# Autodesk Inventor assembly: PowerDistroAssembly_RevB
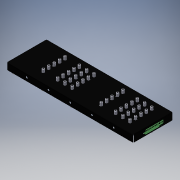
[picture p0: Inventor's stored thumbnail of the model, 180x180]
Saved by Autodesk Inventor 2018 (Build 220112000, 112)
## iProperties
Created: 2018-06-27
Part Number: PowerDistroAssembly_RevB
Document SubType Name: Assembly
Designer: Rich
Author: Rich
## Documents named in this file (8)
- C:\Users\Rich\development\UWaterloo\power-distro.git\SolidModels\PowerDistroAssembly_RevB.iam
- C:\Users\Rich\development\UWaterloo\power-distro.git\SolidModels\power_distro_pcb_RevB.ipt
- C:\Users\Rich\development\UWaterloo\power-distro.git\SolidModels\rcj-021.iam
- C:\Users\Rich\development\UWaterloo\power-distro.git\SolidModels\Enclosure2_RevB_Outer.ipt
- C:\Users\Rich\development\UWaterloo\power-distro.git\SolidModels\Enclosure2_RevB_Inner.ipt
- C:\Users\Rich\development\UWaterloo\power-distro.git\SolidModels\keystone-PN1608-2.ipt
- C:\Users\Rich\development\UWaterloo\power-distro.git\SolidModels\6-32x0.25 Slotted Flathead.ipt
- C:\Users\Rich\development\UWaterloo\power-distro.git\SolidModels\3_5mm_5_08mm_adapter_assembly.iam
## Components (77 placed, 7 different names)
1. power_distro_pcb_RevB:1 — Mate:1, Mate:2, Mate:3, Mate:4, Angle:6, Tangent:1, Mate:5, Angle:7, Mate:6, Mate:7, Mate:10, Mate:11, Mate:12, Mate:13, Mate:14, Mate:15, Mate:16, Mate:17, Mate:18, Mate:19, Mate:20, Mate:21, Mate:22, Mate:23, Mate:24, Mate:25, Mate:26, Mate:27, Insert:1, Insert:2, Insert:3, Insert:4, Insert:5, Insert:6, Insert:7, Insert:8, Insert:9, Mate:34, Mate:35, Mate:36, Mate:37, Mate:38, Mate:39
2. Enclosure2_RevB_Outer:1 — Mate:30, Mate:31, Mate:32
3. Enclosure2_RevB_Inner:2 — Mate:8, Mate:9, Mate:28, Mate:30, Insert:10, Mate:33
4. keystone-PN1608-2:1 — Mate:6, Mate:7, Mate:8, Mate:9
5. keystone-PN1608-2:2 — Mate:10, Mate:27
6. keystone-PN1608-2:3 — Mate:15, Mate:21, Mate:28, Mate:29
7. keystone-PN1608-2:4 — Mate:16, Mate:20
8. keystone-PN1608-2:5 — Mate:11, Mate:25
9. keystone-PN1608-2:6 — Mate:18, Mate:19
10. keystone-PN1608-2:7 — Mate:17, Mate:22
11. keystone-PN1608-2:8 — Mate:14, Mate:26
12. keystone-PN1608-2:9 — Mate:13, Mate:23
13. keystone-PN1608-2:10 — Mate:12, Mate:24
14. 6-32x0.25 Slotted Flathead:1 — Mate:29
15. 6-32x0.25 Slotted Flathead:2 — Insert:1
16. 6-32x0.25 Slotted Flathead:3 — Insert:6
17. 6-32x0.25 Slotted Flathead:4 — Insert:7
18. 6-32x0.25 Slotted Flathead:5 — Insert:8
19. 6-32x0.25 Slotted Flathead:6 — Insert:9
20. 6-32x0.25 Slotted Flathead:7 — Insert:5
21. 6-32x0.25 Slotted Flathead:8 — Insert:4
22. 6-32x0.25 Slotted Flathead:9 — Insert:3
23. 6-32x0.25 Slotted Flathead:10 — Insert:2
24. 6-32x0.25 Slotted Flathead:11
25. 6-32x0.25 Slotted Flathead:12
26. 6-32x0.25 Slotted Flathead:13
27. 6-32x0.25 Slotted Flathead:14
28. 6-32x0.25 Slotted Flathead:15
29. 6-32x0.25 Slotted Flathead:16
30. 6-32x0.25 Slotted Flathead:17
31. 6-32x0.25 Slotted Flathead:18 — Mate:31, Mate:33
32. 6-32x0.25 Slotted Flathead:19 — Mate:32, Insert:10
33. 6-32x0.25 Slotted Flathead:20
34. 6-32x0.25 Slotted Flathead:21
35. 6-32x0.25 Slotted Flathead:22
36. 3_5mm_5_08mm_adapter_assembly:1 [sub-assembly] — Mate:34, Mate:35, Mate:36
37. 3_5mm_5_08mm_adapter_assembly:2 [sub-assembly] — Mate:37, Mate:38, Mate:39
38. rcj-021:2 [sub-assembly] — Mate:4, Angle:6, Tangent:1
39. rcj-021:6 [sub-assembly]
40. rcj-021:10 [sub-assembly]
41. rcj-021:14 [sub-assembly]
42. rcj-021:18 [sub-assembly]
43. rcj-021:22 [sub-assembly]
44. rcj-021:26 [sub-assembly]
45. rcj-021:30 [sub-assembly]
46. rcj-021:34 [sub-assembly]
47. rcj-021:38 [sub-assembly]
48. rcj-021:3 [sub-assembly] — Mate:5, Angle:7
49. rcj-021:4 [sub-assembly]
50. rcj-021:5 [sub-assembly]
51. rcj-021:7 [sub-assembly]
52. rcj-021:8 [sub-assembly]
53. rcj-021:9 [sub-assembly]
54. rcj-021:11 [sub-assembly]
55. rcj-021:12 [sub-assembly]
56. rcj-021:13 [sub-assembly]
57. rcj-021:15 [sub-assembly]
58. rcj-021:16 [sub-assembly]
59. rcj-021:17 [sub-assembly]
60. rcj-021:19 [sub-assembly]
61. rcj-021:20 [sub-assembly]
62. rcj-021:21 [sub-assembly]
63. rcj-021:23 [sub-assembly]
64. rcj-021:24 [sub-assembly]
65. rcj-021:25 [sub-assembly]
66. rcj-021:27 [sub-assembly]
67. rcj-021:28 [sub-assembly]
68. rcj-021:29 [sub-assembly]
69. rcj-021:31 [sub-assembly]
70. rcj-021:32 [sub-assembly]
71. rcj-021:33 [sub-assembly]
72. rcj-021:35 [sub-assembly]
73. rcj-021:36 [sub-assembly]
74. rcj-021:37 [sub-assembly]
75. rcj-021:39 [sub-assembly]
76. rcj-021:40 [sub-assembly]
77. rcj-021:41 [sub-assembly]
## Component patterns: (10 elements, first: rcj-021:2), (3 elements, first: rcj-021:3), Component Pattern 1:2 (3 elements), Component Pattern 1:3 (3 elements), Component Pattern 1:4 (3 elements), Component Pattern 1:5 (3 elements), Component Pattern 1:6 (3 elements), Component Pattern 1:7 (3 elements), Component Pattern 1:8 (3 elements), Component Pattern 1:9 (3 elements), Component Pattern 1:10 (3 elements)
## Relationships (52: Mate 39, Insert 10, Angle 2, Tangent 1)
- Mate:1: power_distro_pcb_RevB:1
- Mate:2: power_distro_pcb_RevB:1
- Mate:3: power_distro_pcb_RevB:1
- Mate:4: power_distro_pcb_RevB:1 ↔ rcj-021:2
- Angle:6 (0 deg): power_distro_pcb_RevB:1 ↔ rcj-021:2
- Tangent:1: power_distro_pcb_RevB:1 ↔ rcj-021:2
- Mate:5: power_distro_pcb_RevB:1 ↔ rcj-021:3
- Angle:7 (0 deg): power_distro_pcb_RevB:1 ↔ rcj-021:3
- Mate:6: power_distro_pcb_RevB:1 ↔ keystone-PN1608-2:1
- Mate:7: power_distro_pcb_RevB:1 ↔ keystone-PN1608-2:1
- Mate:8: Enclosure2_RevB_Inner:2 ↔ keystone-PN1608-2:1
- Mate:9: Enclosure2_RevB_Inner:2 ↔ keystone-PN1608-2:1
- Mate:10: power_distro_pcb_RevB:1 ↔ keystone-PN1608-2:2
- Mate:11: power_distro_pcb_RevB:1 ↔ keystone-PN1608-2:5
- Mate:12: power_distro_pcb_RevB:1 ↔ keystone-PN1608-2:10
- Mate:13: power_distro_pcb_RevB:1 ↔ keystone-PN1608-2:9
- Mate:14: power_distro_pcb_RevB:1 ↔ keystone-PN1608-2:8
- Mate:15: power_distro_pcb_RevB:1 ↔ keystone-PN1608-2:3
- Mate:16: power_distro_pcb_RevB:1 ↔ keystone-PN1608-2:4
- Mate:17: power_distro_pcb_RevB:1 ↔ keystone-PN1608-2:7
- Mate:18: power_distro_pcb_RevB:1 ↔ keystone-PN1608-2:6
- Mate:19: power_distro_pcb_RevB:1 ↔ keystone-PN1608-2:6
- Mate:20: power_distro_pcb_RevB:1 ↔ keystone-PN1608-2:4
- Mate:21: power_distro_pcb_RevB:1 ↔ keystone-PN1608-2:3
- Mate:22: power_distro_pcb_RevB:1 ↔ keystone-PN1608-2:7
- Mate:23: power_distro_pcb_RevB:1 ↔ keystone-PN1608-2:9
- Mate:24: power_distro_pcb_RevB:1 ↔ keystone-PN1608-2:10
- Mate:25: power_distro_pcb_RevB:1 ↔ keystone-PN1608-2:5
- Mate:26: power_distro_pcb_RevB:1 ↔ keystone-PN1608-2:8
- Mate:27: power_distro_pcb_RevB:1 ↔ keystone-PN1608-2:2
- Mate:28: Enclosure2_RevB_Inner:2 ↔ keystone-PN1608-2:3
- Mate:29: keystone-PN1608-2:3 ↔ 6-32x0.25 Slotted Flathead:1
- Insert:1: power_distro_pcb_RevB:1 ↔ 6-32x0.25 Slotted Flathead:2
- Insert:2: power_distro_pcb_RevB:1 ↔ 6-32x0.25 Slotted Flathead:10
- Insert:3: power_distro_pcb_RevB:1 ↔ 6-32x0.25 Slotted Flathead:9
- Insert:4: power_distro_pcb_RevB:1 ↔ 6-32x0.25 Slotted Flathead:8
- Insert:5: power_distro_pcb_RevB:1 ↔ 6-32x0.25 Slotted Flathead:7
- Insert:6: power_distro_pcb_RevB:1 ↔ 6-32x0.25 Slotted Flathead:3
- Insert:7: power_distro_pcb_RevB:1 ↔ 6-32x0.25 Slotted Flathead:4
- Insert:8: power_distro_pcb_RevB:1 ↔ 6-32x0.25 Slotted Flathead:5
- Insert:9: power_distro_pcb_RevB:1 ↔ 6-32x0.25 Slotted Flathead:6
- Mate:30: Enclosure2_RevB_Outer:1 ↔ Enclosure2_RevB_Inner:2
- Mate:31: Enclosure2_RevB_Outer:1 ↔ 6-32x0.25 Slotted Flathead:18
- Mate:32: Enclosure2_RevB_Outer:1 ↔ 6-32x0.25 Slotted Flathead:19
- Insert:10: Enclosure2_RevB_Inner:2 ↔ 6-32x0.25 Slotted Flathead:19
- Mate:33: Enclosure2_RevB_Inner:2 ↔ 6-32x0.25 Slotted Flathead:18
- Mate:34: power_distro_pcb_RevB:1 ↔ 3_5mm_5_08mm_adapter_assembly:1
- Mate:35: power_distro_pcb_RevB:1 ↔ 3_5mm_5_08mm_adapter_assembly:1
- Mate:36: power_distro_pcb_RevB:1 ↔ 3_5mm_5_08mm_adapter_assembly:1
- Mate:37: power_distro_pcb_RevB:1 ↔ 3_5mm_5_08mm_adapter_assembly:2
- Mate:38: power_distro_pcb_RevB:1 ↔ 3_5mm_5_08mm_adapter_assembly:2
- Mate:39: power_distro_pcb_RevB:1 ↔ 3_5mm_5_08mm_adapter_assembly:2
